# Autodesk Inventor assembly: gantry_frame
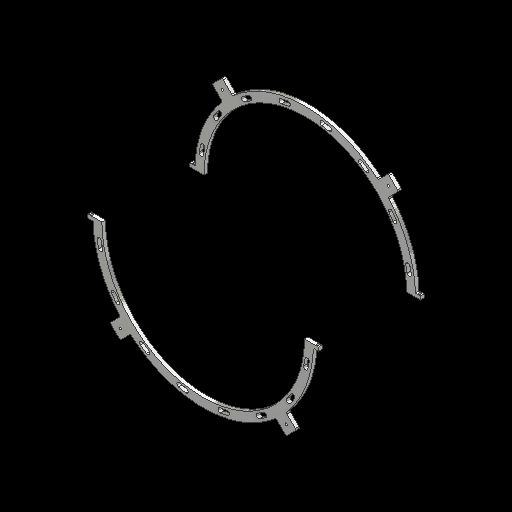
[picture p0: Inventor's stored thumbnail of the model, 512x512]
Saved by Autodesk Inventor 2026.1 (Build 301233000, 233)
## iProperties
Created: 2025-09-18
Part Number: gantry_frame
Document SubType Name: Assembly
Designer: drago
Author: drago
## Documents named in this file (2)
- C:\Users\drago\Desktop\_QIST4500_Multidisciplinary_Team_Project\Proteox MX magnet positioner CAD\gantry_frame\full_ring.iam
- C:\Users\drago\Desktop\_QIST4500_Multidisciplinary_Team_Project\Proteox MX magnet positioner CAD\gantry_frame\half_ring.ipt
## Components (2 placed, 1 different names)
1. half_ring:1 — Mate:1, Mate:2
2. half_ring:2
## Relationships (2: Mate 2)
- Mate:1: half_ring:1
- Mate:2: half_ring:1
